# Autodesk Inventor assembly: Battery_Clip_R
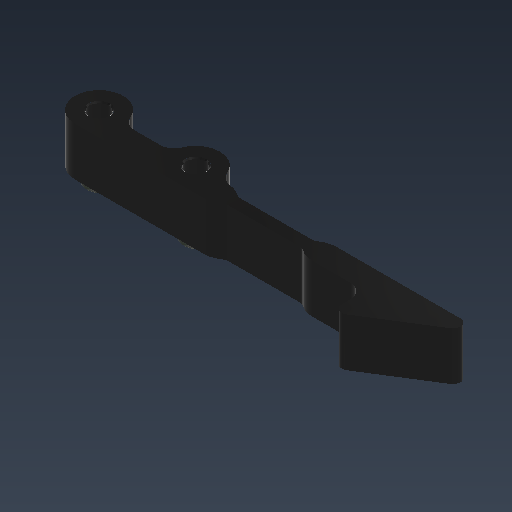
[picture p0: Inventor's stored thumbnail of the model, 512x512]
Saved by Autodesk Inventor 2024.1 (Build 281209000, 209)
## iProperties
Created: 2023-12-07
Part Number: Battery_Clip_R
Document SubType Name: Assembly
Designer: dzw04
Mass: 6.842 g
Surface Area: 34.9347 cm^2
Volume: 4.73196 cm^3
Density: 1.44591 g/cm^3
Author: dzw04
## Documents named in this file (5)
- C:\Users\dzw04\Saxion\Mechatronica Lectoraat LMECH LED - Database ARG\Component_Database\SARAX\01. CAD\01. 3D_Drawing\02. Sub_Assemblies\Battery_Tray\02. Sub_Assemblies\Battery_Clip_R.iam
- C:\Users\dzw04\Saxion\Mechatronica Lectoraat LMECH LED - Database ARG\Component_Database\SARAX\01. CAD\01. 3D_Drawing\02. Sub_Assemblies\Battery_Tray\01. Parts\Battery_Clip.ipt
- C:\Users\dzw04\Saxion\Mechatronica Lectoraat LMECH LED - Database ARG\Component_Database\SARAX\01. CAD\01. 3D_Drawing\01. Parts\Threaded_Insert_M3x4.ipt
- C:\Users\dzw04\Saxion\Mechatronica Lectoraat LMECH LED - Database ARG\Component_Database\SARAX\01. CAD\01. 3D_Drawing\01. Parts\en-US\ISO 7380-1\ISO 7380-1 - M3 x 8.ipt
- C:\Users\dzw04\Saxion\Mechatronica Lectoraat LMECH LED - Database ARG\Component_Database\SARAX\01. CAD\01. 3D_Drawing\Parameters.xlsx
## Components (5 placed, 3 different names)
1. Battery_Clip:1 — Mate:1, Mate:2, Flush:1, Flush:2, Mate:3, Mate:5
2. Threaded_Insert_M3x4:1 — Mate:1, Flush:2, Mate:6
3. Threaded_Insert_M3x4:2 — Mate:2, Flush:1, Mate:4
4. ISO 7380-1 M3 x 8:1 — Mate:5, Mate:6
5. ISO 7380-1 M3 x 8:2 — Mate:3, Mate:4
## Relationships (8: Mate 6, Flush 2)
- Mate:1: Battery_Clip:1 ↔ Threaded_Insert_M3x4:1
- Mate:2: Battery_Clip:1 ↔ Threaded_Insert_M3x4:2
- Flush:1: Battery_Clip:1 ↔ Threaded_Insert_M3x4:2
- Flush:2: Battery_Clip:1 ↔ Threaded_Insert_M3x4:1
- Mate:3 (2 mm): Battery_Clip:1 ↔ ISO 7380-1 M3 x 8:2
- Mate:4: Threaded_Insert_M3x4:2 ↔ ISO 7380-1 M3 x 8:2
- Mate:5 (2 mm): Battery_Clip:1 ↔ ISO 7380-1 M3 x 8:1
- Mate:6: Threaded_Insert_M3x4:1 ↔ ISO 7380-1 M3 x 8:1
## Named parameters: NumberOfArms = 4, RotorToRotor = 900 mm, MountToMotorCenter = 0 mm, ArmPosition = 5 deg, LoadpipeLength = 450 mm, NumberOfBatterys = 2, BatteryLength = 200 mm, BatteryWidth = 62 mm, BatteryHeight = 76 mm, ThicknessBodyOuterPlate = 2 mm, ThicknessBodyCenterPlate = 2 mm, ThicknessLegLoadpipePlate = 2 mm, ThicknessBatteryTray = 2 mm, ThicknessBatteryTopTray = 1 mm, LandingGearHeight = 400 mm, LandingGearStabilityBar = 525 mm, LandingGearRod = 390 mm, StartAngleArm = 45 deg, MotorMountCenter = 71.5 mm
